# Autodesk Inventor assembly: Сборка1
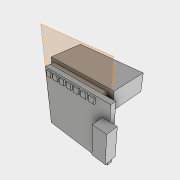
[picture p0: Inventor's stored thumbnail of the model, 180x180]
Saved by Autodesk Inventor 2021.2 (Build 252289000, 289)
## iProperties
Created: 2025-10-22
Part Number: Сборка1
Document SubType Name: Assembly
Designer: Захаров
Author: Захаров
## Documents named in this file (4)
- C:\Users\User\Documents\ARHeadGen1\Сборка1.iam
- C:\Users\User\Documents\ARHeadGen1\ЛЦМК.00002.00.00.00.00.01.ipt
- C:\Users\User\Documents\ARHeadGen1\ЛЦМК000002.00.00.00.00.02.ipt
- C:\Users\User\Documents\ARHeadGen1\ЛЦМК0000002.00.00.00.00.03.ipt
## Components (3 placed, 3 different names)
1. ЛЦМК.00002.00.00.00.00.01:1 — Совмещение:1
2. ЛЦМК000002.00.00.00.00.02:1
3. ЛЦМК0000002.00.00.00.00.03:1 — Совмещение:1
## Relationships (1: Mate 1)
- Совмещение:1 [Mate]: ЛЦМК.00002.00.00.00.00.01:1 ↔ ЛЦМК0000002.00.00.00.00.03:1
